# Autodesk Inventor assembly: elevator
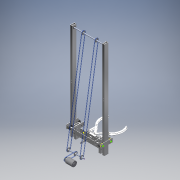
[picture p0: Inventor's stored thumbnail of the model, 180x180]
Saved by Autodesk Inventor 2017 (Build 210142000, 142)
## iProperties
Created: 2017-12-27
Part Number: elevator
Document SubType Name: Assembly
Designer: Micah
Mass: 4635.04 g
Surface Area: 10973.2 cm^2
Volume: 1751.48 cm^3
Density: 2.64636 g/cm^3
Author: Micah
## Documents named in this file (10)
- C:\Users\Micah\Desktop\inventor\CADathon-2017\2AM-17-A-0200 - Smokestack Elevator\2AM-17-A-0200 - elevator.iam
- C:\Users\Micah\Desktop\inventor\CADathon-2017\2AM-17-A-0200 - Smokestack Elevator\2AM-17-P-0201 - main structure.ipt
- C:\Users\Micah\Desktop\inventor\CADathon-2017\2AM-17-A-0200 - Smokestack Elevator\COTS\0_500_Hex_ID_x_1_125_OD_x_0_313_WD_Flanged_Bearing_v2_217-3875.ipt
- C:\Users\Micah\Desktop\inventor\CADathon-2017\2AM-17-A-0200 - Smokestack Elevator\2AM-17-P-0204 - top hex shaft.ipt
- C:\Users\Micah\Desktop\inventor\CADathon-2017\2AM-17-A-0200 - Smokestack Elevator\COTS\217-2737.20121205.ipt
- C:\Users\Micah\Desktop\inventor\CADathon-2017\2AM-17-A-0200 - Smokestack Elevator\2AM-17-A-1200 - moving part.iam
- C:\Users\Micah\Desktop\inventor\CADathon-2017\2AM-17-A-0200 - Smokestack Elevator\2AM-17-A-5200 - claw.iam
- C:\Users\Micah\Desktop\inventor\CADathon-2017\2AM-17-A-0200 - Smokestack Elevator\2AM-17-A-7200 - slider motor and gearbox.iam
- C:\Users\Micah\Desktop\inventor\CADathon-2017\2AM-17-A-0200 - Smokestack Elevator\2AM-17-A-0200 - elevator\Design Accelerator\Chain Drive1.iam
- C:\Users\Micah\Desktop\inventor\CADathon-2017\2AM-17-A-0200 - Smokestack Elevator\2AM-17-A-0200 - elevator\Design Accelerator\Chain Drive2.iam
## Components (12 placed, 8 different names)
1. 2AM-17-P-0201 - main structure:2 — Mate:4
2. 2AM-17-P-0201 - main structure:3 — Mate:5, Mate:7
3. 0_500_Hex_ID_x_1_125_OD_x_0_313_WD_Flanged_Bearing_v2_217-3875:1 — Mate:4, Rigid:1
4. 0_500_Hex_ID_x_1_125_OD_x_0_313_WD_Flanged_Bearing_v2_217-3875:2 — Mate:5
5. 2AM-17-P-0204 - top hex shaft:1 — Rigid:1, Rigid:2, Rigid:3
6. 217-2737.20121205:1 — Rigid:2
7. 217-2737.20121205:2 — Rigid:3
8. 2AM-17-A-1200 - moving part:1 [sub-assembly] — Mate:7, Mate:8, Mate:9
9. 2AM-17-A-5200 - claw:1 [sub-assembly] — Mate:8, Mate:9
10. 2AM-17-A-7200 - slider motor and gearbox:1 [sub-assembly]
11. Chain Drive:1 [sub-assembly]
12. Chain Drive:2 [sub-assembly]
## Relationships (8: Mate 5, WeldJoint 3)
- Mate:4: 2AM-17-P-0201 - main structure:2 ↔ 0_500_Hex_ID_x_1_125_OD_x_0_313_WD_Flanged_Bearing_v2_217-3875:1
- Mate:5: 2AM-17-P-0201 - main structure:3 ↔ 0_500_Hex_ID_x_1_125_OD_x_0_313_WD_Flanged_Bearing_v2_217-3875:2
- Rigid:1 [WeldJoint] (-14.2875 mm): 0_500_Hex_ID_x_1_125_OD_x_0_313_WD_Flanged_Bearing_v2_217-3875:1 ↔ 2AM-17-P-0204 - top hex shaft:1
- Rigid:2 [WeldJoint]: 2AM-17-P-0204 - top hex shaft:1 ↔ 217-2737.20121205:1
- Rigid:3 [WeldJoint]: 2AM-17-P-0204 - top hex shaft:1 ↔ 217-2737.20121205:2
- Mate:7: 2AM-17-P-0201 - main structure:3 ↔ 2AM-17-A-1200 - moving part:1
- Mate:8: 2AM-17-A-1200 - moving part:1 ↔ 2AM-17-A-5200 - claw:1
- Mate:9: 2AM-17-A-1200 - moving part:1 ↔ 2AM-17-A-5200 - claw:1
